# Autodesk Inventor assembly: GL5528-Photoresistor
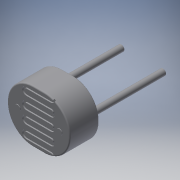
[picture p0: Inventor's stored thumbnail of the model, 180x180]
Saved by Autodesk Inventor 2016 (Build 200138000, 138)
## iProperties
Company: ksu MCAD
Created: 2017-09-24
Part Number: GL5528-Photoresistor
Description: FreeCAD Model
Document SubType Name: Assembly
Designer: Luke
Authority: Unknown
Sending System: FreeCAD
Preprocessor: Open CASCADE STEP processor 6.9
Title: /home/erik/kicad/libraries/parts_erik.3dshapes/GL5528-Photoresistor.step
Author: kicad StepUp
## Documents named in this file (2)
- E:\CURRENT\PROJECTS\POMODORO\Mechanical\Parts\Standard\Photoresistor\GL5528-Photoresistor.iam
- E:\CURRENT\PROJECTS\POMODORO\Mechanical\Parts\Standard\Photoresistor\GL5528-Photoresistor.ipt
## Components (1 placed, 1 different names)
1. 1 — Flush:1
## Relationships (1: Flush 1)
- Flush:1 (-6.5 mm): 1
